# Autodesk Inventor assembly: Traction Wheel Assembly 1764
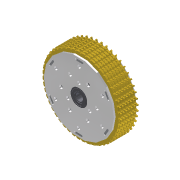
[picture p0: Inventor's stored thumbnail of the model, 180x180]
Saved by Autodesk Inventor 2011 (Build 150239000, 239)
## iProperties
Created: 2010-01-11
Part Number: Traction Wheel Assembly 1764
Document SubType Name: Assembly
Designer: wbridges
Author: wbridges
## Documents named in this file (5)
- R:\2010-2011\CMO\Web Site\CADalog\Wheels\Small Traction Wheel 1764\Traction Wheel Assembly 1764.iam
- R:\2010-2011\CMO\Web Site\CADalog\Wheels\Small Traction Wheel 1764\Traction Wheel Side Plate 1764.ipt
- R:\2010-2011\CMO\Web Site\CADalog\Wheels\Small Traction Wheel 1764\Lateral Wheel Casing 1764.ipt
- R:\2010-2011\CMO\Web Site\CADalog\Wheels\Small Traction Wheel 1764\Traction Tread 1764.ipt
- R:\2010-2011\CMO\Web Site\CADalog\Wheels\Small Traction Wheel 1764\Wheel Bearing 1764\Wheel Bearing 1764.iam
## Components (8 placed, 4 different names)
1. Traction Wheel Side Plate 1764:1 — Flush:2, Mate:1, Mate:4, Mate:5, Mate:7, Mate:8, Mate:9, Mate:10, Flush:7
2. Traction Wheel Side Plate 1764:2 — Flush:2, Mate:1, Mate:6, Flush:8
3. Lateral Wheel Casing 1764:1 — Mate:2, Flush:3, Flush:4, Mate:3, Flush:5, Flush:6, Mate:4, Mate:5, Mate:6
4. Lateral Wheel Casing 1764:2 — Mate:2, Flush:3, Flush:4, Mate:7
5. Lateral Wheel Casing 1764:3 — Mate:3, Flush:5, Flush:6
6. Traction Tread 1764:1 — Mate:8, Mate:9
7. Wheel Bearing 1764:1 [sub-assembly] — Mate:10, Flush:7, Mate:11
8. Wheel Bearing 1764:2 [sub-assembly] — Mate:11, Flush:8
## Relationships (18: Mate 11, Flush 7)
- Flush:2: Traction Wheel Side Plate 1764:1 ↔ Traction Wheel Side Plate 1764:2
- Mate:1: Traction Wheel Side Plate 1764:1 ↔ Traction Wheel Side Plate 1764:2
- Mate:2: Lateral Wheel Casing 1764:1 ↔ Lateral Wheel Casing 1764:2
- Flush:3: Lateral Wheel Casing 1764:1 ↔ Lateral Wheel Casing 1764:2
- Flush:4: Lateral Wheel Casing 1764:1 ↔ Lateral Wheel Casing 1764:2
- Mate:3: Lateral Wheel Casing 1764:1 ↔ Lateral Wheel Casing 1764:3
- Flush:5: Lateral Wheel Casing 1764:1 ↔ Lateral Wheel Casing 1764:3
- Flush:6: Lateral Wheel Casing 1764:1 ↔ Lateral Wheel Casing 1764:3
- Mate:4: Traction Wheel Side Plate 1764:1 ↔ Lateral Wheel Casing 1764:1
- Mate:5: Traction Wheel Side Plate 1764:1 ↔ Lateral Wheel Casing 1764:1
- Mate:6: Traction Wheel Side Plate 1764:2 ↔ Lateral Wheel Casing 1764:1
- Mate:7: Traction Wheel Side Plate 1764:1 ↔ Lateral Wheel Casing 1764:2
- Mate:8: Traction Wheel Side Plate 1764:1 ↔ Traction Tread 1764:1
- Mate:9: Traction Wheel Side Plate 1764:1 ↔ Traction Tread 1764:1
- Mate:10: Traction Wheel Side Plate 1764:1 ↔ Wheel Bearing 1764:1
- Flush:7: Traction Wheel Side Plate 1764:1 ↔ Wheel Bearing 1764:1
- Mate:11: Wheel Bearing 1764:1 ↔ Wheel Bearing 1764:2
- Flush:8: Traction Wheel Side Plate 1764:2 ↔ Wheel Bearing 1764:2
